# Autodesk Inventor assembly: Spigot Short
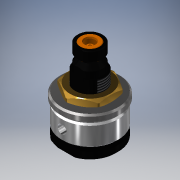
[picture p0: Inventor's stored thumbnail of the model, 180x180]
Saved by Autodesk Inventor 2019 (Build 230136000, 136)
## iProperties
Created: 2018-04-22
Part Number: Spigot Short
Document SubType Name: Assembly
Designer: IEUser
Author: IEUser
## Documents named in this file (6)
- C:\Users\IEUser\Desktop\lrut-inflatable-ring-standard-master\Spigots\Spigot Short.iam
- C:\Users\IEUser\Desktop\lrut-inflatable-ring-standard-master\Spigots\Spigot Short.ipt
- C:\Users\IEUser\Desktop\lrut-inflatable-ring-standard-master\Spigots\Spacer.ipt
- C:\Users\IEUser\Desktop\lrut-inflatable-ring-standard-master\Stock Components\Accu Group\HPCW-M10-A4.ipt
- C:\Users\IEUser\Desktop\lrut-inflatable-ring-standard-master\Stock Components\Elma Electronic\4024-86.ipt
- C:\Users\IEUser\Desktop\lrut-inflatable-ring-standard-master\Stock Components\Amphenol\252124.ipt
## Components (5 placed, 5 different names)
1. Spigot Short:1 — Mate:1, Mate:2, Mate:4, Mate:6, Insert:1
2. Spacer:1 — Mate:1, Mate:2, Mate:3
3. HPCW-M10-A4:1 — Mate:3, Mate:4, Mate:5
4. 4024-86:1 — Mate:5, Mate:6
5. 252124:1 — Insert:1
## Relationships (7: Mate 6, Insert 1)
- Mate:1: Spigot Short:1 ↔ Spacer:1
- Mate:2: Spigot Short:1 ↔ Spacer:1
- Mate:3 (1 mm): Spacer:1 ↔ HPCW-M10-A4:1
- Mate:4: Spigot Short:1 ↔ HPCW-M10-A4:1
- Mate:5: HPCW-M10-A4:1 ↔ 4024-86:1
- Mate:6: Spigot Short:1 ↔ 4024-86:1
- Insert:1: Spigot Short:1 ↔ 252124:1
